# Autodesk Inventor assembly: przegub_1
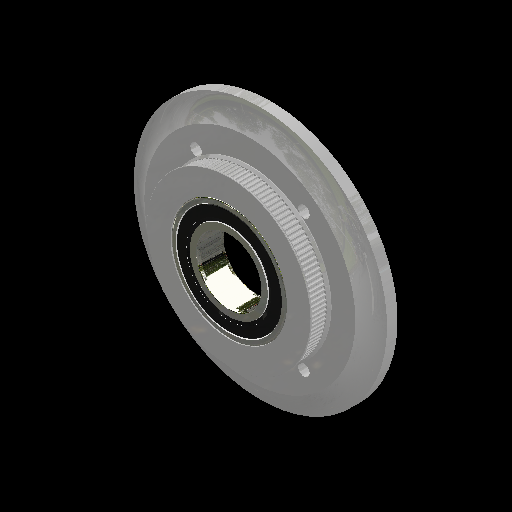
[picture p0: Inventor's stored thumbnail of the model, 512x512]
Saved by Autodesk Inventor 2024.4 (Build 284460000, 460)
## iProperties
Created: 2025-10-04
Part Number: przegub_1
Document SubType Name: Assembly
Designer: User
Mass: 113.482 g
Surface Area: 478.278 cm^2
Volume: 113.482 cm^3
Density: 1 g/cm^3
Author: User
## Documents named in this file (5)
- C:\Users\Duszy\Desktop\Projekty\Dummy\Dummy_v2\Model\Model\przegub_1\przegub_0.iam
- C:\Users\Duszy\Desktop\Projekty\Dummy\Dummy_v2\Model\Model\przegub_1\6661K89_Ball Bearing.ipt
- C:\Users\Duszy\Desktop\Projekty\Dummy\Dummy_v2\Model\Model\przegub_1\podstawa_platforma.ipt
- C:\Users\Duszy\Desktop\Projekty\Dummy\Dummy_v2\Model\Model\modele_gotowe\Modele_elementów\94459A150_Heat-Set Inserts for Plastic.ipt
- C:\Users\Duszy\Desktop\Projekty\Dummy\Dummy_v2\Model\Model\modele_gotowe\Modele_elementów\90258A214_Phillips Oval Head Screws.ipt
## Components (10 placed, 4 different names)
1. 6661K89_Ball Bearing:1 — Obrotowe:14
2. podstawa_platforma:1 — Obrotowe:10, Obrotowe:11, Obrotowe:12, Obrotowe:13, Obrotowe:14
3. 94459A150_Heat-Set Inserts for Plastic:1 — Obrotowe:3, Obrotowe:10
4. 90258A214_Phillips Oval Head Screws:1 — Obrotowe:3
5. 94459A150_Heat-Set Inserts for Plastic:2 — Obrotowe:13
6. 90258A214_Phillips Oval Head Screws:2
7. 94459A150_Heat-Set Inserts for Plastic:3 — Obrotowe:12
8. 90258A214_Phillips Oval Head Screws:3
9. 94459A150_Heat-Set Inserts for Plastic:4 — Obrotowe:11
10. 90258A214_Phillips Oval Head Screws:4
## Relationships (9: RevoluteJoint 9)
- Obrotowe:3 [RevoluteJoint] (-5 mm): 94459A150_Heat-Set Inserts for Plastic:1 ↔ 90258A214_Phillips Oval Head Screws:1
- [RevoluteJoint] (-5 mm): 94459A150_Heat-Set Inserts for Plastic:2 ↔ 90258A214_Phillips Oval Head Screws:2
- [RevoluteJoint] (-5 mm): 94459A150_Heat-Set Inserts for Plastic:3 ↔ 90258A214_Phillips Oval Head Screws:3
- [RevoluteJoint] (-5 mm): 94459A150_Heat-Set Inserts for Plastic:4 ↔ 90258A214_Phillips Oval Head Screws:4
- Obrotowe:10 [RevoluteJoint] (0.1 mm): podstawa_platforma:1 ↔ 94459A150_Heat-Set Inserts for Plastic:1
- Obrotowe:11 [RevoluteJoint] (0.1 mm): podstawa_platforma:1 ↔ 94459A150_Heat-Set Inserts for Plastic:4
- Obrotowe:12 [RevoluteJoint] (0.1 mm): podstawa_platforma:1 ↔ 94459A150_Heat-Set Inserts for Plastic:3
- Obrotowe:13 [RevoluteJoint] (0.1 mm): podstawa_platforma:1 ↔ 94459A150_Heat-Set Inserts for Plastic:2
- Obrotowe:14 [RevoluteJoint] (-12.32 mm): 6661K89_Ball Bearing:1 ↔ podstawa_platforma:1
## Named parameters: d10_d8 = -5 mm, d11_d9 = 0 deg, d12_d8 = -5 mm, d13_d9 = 0 deg, d14_d8 = -5 mm, d15_d9 = 0 deg
